# Autodesk Inventor assembly: smble_zona_calor
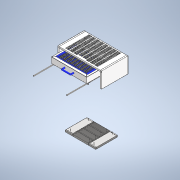
[picture p0: Inventor's stored thumbnail of the model, 180x180]
Saved by Autodesk Inventor 2021 (Build 250183000, 183)
## iProperties
Created: 2021-04-15
Part Number: smble_zona_calor
Document SubType Name: Assembly
Designer: Leonardo Fabio Mercado Benítez
Author: Leonardo Fabio Mercado Benítez
## Documents named in this file (10)
- C:\Users\leo7s\Documents\Universidad\04 PAI\03 Proyecto\03 Repositorio\Proyecto_PAI_2021\01 CAD\smble_zona_calor.iam
- C:\Users\leo7s\Documents\Universidad\04 PAI\03 Proyecto\03 Repositorio\Proyecto_PAI_2021\01 CAD\Ensamblaje carcasa superior.iam
- C:\Users\leo7s\Documents\Universidad\04 PAI\03 Proyecto\03 Repositorio\Proyecto_PAI_2021\01 CAD\soporte_inferior_zona_calor.ipt
- C:\Users\leo7s\Documents\Universidad\04 PAI\03 Proyecto\03 Repositorio\Proyecto_PAI_2021\01 CAD\tapa_caja_calor.ipt
- C:\Users\leo7s\Documents\Universidad\04 PAI\03 Proyecto\03 Repositorio\Proyecto_PAI_2021\01 CAD\angulo_caja_calor.ipt
- C:\Users\leo7s\Documents\Universidad\04 PAI\03 Proyecto\03 Repositorio\Proyecto_PAI_2021\01 CAD\buje_carro_zona_calor.ipt
- C:\Users\leo7s\Documents\Universidad\04 PAI\03 Proyecto\03 Repositorio\Proyecto_PAI_2021\01 CAD\barra.ipt
- C:\Users\leo7s\Documents\Universidad\04 PAI\03 Proyecto\03 Repositorio\Proyecto_PAI_2021\01 CAD\mango_zona_calor.ipt
- C:\Users\leo7s\Documents\Universidad\04 PAI\03 Proyecto\03 Repositorio\Proyecto_PAI_2021\01 CAD\resistencia_cuarzo_550W.ipt
- C:\Users\leo7s\Documents\Universidad\04 PAI\03 Proyecto\03 Repositorio\Proyecto_PAI_2021\01 CAD\resistencia_cuarzo_250-300W.ipt
## Components (18 placed, 9 different names)
1. Ensamblaje carcasa superior:1 [sub-assembly] — Coincidencia:1, Coincidencia:2, Coincidencia:11, Coincidencia:12
2. soporte_inferior_zona_calor:1 — Coincidencia:1, Coincidencia:2, Coincidencia:3, Nivelación:1, Nivelación:2, Coincidencia:5, Nivelación:3, Nivelación:4, Coincidencia:6, Nivelación:5, Nivelación:6, Coincidencia:15, Insertar:5, Insertar:6
3. tapa_caja_calor:1 — Coincidencia:3, Nivelación:1, Nivelación:2
4. angulo_caja_calor:1 — Coincidencia:5, Nivelación:3, Nivelación:4, Coincidencia:7, Coincidencia:8, Insertar:1, Insertar:2
5. angulo_caja_calor:2 — Coincidencia:6, Nivelación:5, Nivelación:6, Coincidencia:9, Coincidencia:10, Insertar:3, Insertar:4
6. buje_carro_zona_calor:1 — Coincidencia:9, Insertar:3
7. buje_carro_zona_calor:2 — Coincidencia:8, Insertar:2, Coincidencia:14
8. buje_carro_zona_calor:3 — Coincidencia:10, Insertar:4
9. buje_carro_zona_calor:4 — Coincidencia:7, Insertar:1, Coincidencia:13
10. barra:1 — Coincidencia:11, Coincidencia:13
11. barra:2 — Coincidencia:12, Coincidencia:14
12. mango_zona_calor:1 — Coincidencia:15, Insertar:5, Insertar:6
13. resistencia_cuarzo_550W:1 — Nivelación:7, Nivelación:8, Nivelación:9, Nivelación:10, Nivelación:11, Coincidencia:16, Nivelación:12, Nivelación:13, Coincidencia:17, Coincidencia:18, Coincidencia:19
14. resistencia_cuarzo_550W:2 — Nivelación:7, Coincidencia:22, Nivelación:14
15. resistencia_cuarzo_250-300W:1 — Nivelación:8, Coincidencia:17, Coincidencia:21
16. resistencia_cuarzo_250-300W:2 — Nivelación:11, Nivelación:13, Coincidencia:19, Coincidencia:21, Coincidencia:22, Nivelación:14
17. resistencia_cuarzo_250-300W:3 — Nivelación:9, Coincidencia:18, Coincidencia:20
18. resistencia_cuarzo_250-300W:4 — Nivelación:10, Coincidencia:16, Nivelación:12, Coincidencia:20
## Relationships (41: Mate 21, Flush 14, Insert 6)
- Coincidencia:1 [Mate] (61.24 mm): Ensamblaje carcasa superior:1 ↔ soporte_inferior_zona_calor:1
- Coincidencia:2 [Mate] (29 mm): Ensamblaje carcasa superior:1 ↔ soporte_inferior_zona_calor:1
- Coincidencia:3 [Mate]: soporte_inferior_zona_calor:1 ↔ tapa_caja_calor:1
- Nivelación:1 [Flush] (25.4 mm): soporte_inferior_zona_calor:1 ↔ tapa_caja_calor:1
- Nivelación:2 [Flush] (35.6 mm): soporte_inferior_zona_calor:1 ↔ tapa_caja_calor:1
- Coincidencia:5 [Mate]: soporte_inferior_zona_calor:1 ↔ angulo_caja_calor:1
- Nivelación:3 [Flush]: soporte_inferior_zona_calor:1 ↔ angulo_caja_calor:1
- Nivelación:4 [Flush] (25.4 mm): soporte_inferior_zona_calor:1 ↔ angulo_caja_calor:1
- Coincidencia:6 [Mate]: soporte_inferior_zona_calor:1 ↔ angulo_caja_calor:2
- Nivelación:5 [Flush]: soporte_inferior_zona_calor:1 ↔ angulo_caja_calor:2
- Nivelación:6 [Flush]: soporte_inferior_zona_calor:1 ↔ angulo_caja_calor:2
- Coincidencia:7 [Mate]: angulo_caja_calor:1 ↔ buje_carro_zona_calor:4
- Coincidencia:8 [Mate]: angulo_caja_calor:1 ↔ buje_carro_zona_calor:2
- Coincidencia:9 [Mate]: angulo_caja_calor:2 ↔ buje_carro_zona_calor:1
- Coincidencia:10 [Mate]: angulo_caja_calor:2 ↔ buje_carro_zona_calor:3
- Insertar:1: angulo_caja_calor:1 ↔ buje_carro_zona_calor:4
- Insertar:2: angulo_caja_calor:1 ↔ buje_carro_zona_calor:2
- Insertar:3: angulo_caja_calor:2 ↔ buje_carro_zona_calor:1
- Insertar:4: angulo_caja_calor:2 ↔ buje_carro_zona_calor:3
- Coincidencia:11 [Mate]: Ensamblaje carcasa superior:1 ↔ barra:1
- Coincidencia:12 [Mate]: Ensamblaje carcasa superior:1 ↔ barra:2
- Coincidencia:13 [Mate]: buje_carro_zona_calor:4 ↔ barra:1
- Coincidencia:14 [Mate]: buje_carro_zona_calor:2 ↔ barra:2
- Coincidencia:15 [Mate]: soporte_inferior_zona_calor:1 ↔ mango_zona_calor:1
- Insertar:5: soporte_inferior_zona_calor:1 ↔ mango_zona_calor:1
- Insertar:6: soporte_inferior_zona_calor:1 ↔ mango_zona_calor:1
- Nivelación:7 [Flush]: resistencia_cuarzo_550W:1 ↔ resistencia_cuarzo_550W:2
- Nivelación:8 [Flush]: resistencia_cuarzo_550W:1 ↔ resistencia_cuarzo_250-300W:1
- Nivelación:9 [Flush]: resistencia_cuarzo_550W:1 ↔ resistencia_cuarzo_250-300W:3
- Nivelación:10 [Flush]: resistencia_cuarzo_550W:1 ↔ resistencia_cuarzo_250-300W:4
- Nivelación:11 [Flush]: resistencia_cuarzo_550W:1 ↔ resistencia_cuarzo_250-300W:2
- Coincidencia:16 [Mate]: resistencia_cuarzo_550W:1 ↔ resistencia_cuarzo_250-300W:4
- Nivelación:12 [Flush]: resistencia_cuarzo_550W:1 ↔ resistencia_cuarzo_250-300W:4
- Nivelación:13 [Flush]: resistencia_cuarzo_550W:1 ↔ resistencia_cuarzo_250-300W:2
- Coincidencia:17 [Mate]: resistencia_cuarzo_550W:1 ↔ resistencia_cuarzo_250-300W:1
- Coincidencia:18 [Mate]: resistencia_cuarzo_550W:1 ↔ resistencia_cuarzo_250-300W:3
- Coincidencia:19 [Mate]: resistencia_cuarzo_550W:1 ↔ resistencia_cuarzo_250-300W:2
- Coincidencia:20 [Mate] (11.67 mm): resistencia_cuarzo_250-300W:3 ↔ resistencia_cuarzo_250-300W:4
- Coincidencia:21 [Mate] (11.67 mm): resistencia_cuarzo_250-300W:1 ↔ resistencia_cuarzo_250-300W:2
- Coincidencia:22 [Mate]: resistencia_cuarzo_550W:2 ↔ resistencia_cuarzo_250-300W:2
- Nivelación:14 [Flush]: resistencia_cuarzo_550W:2 ↔ resistencia_cuarzo_250-300W:2
